# Autodesk Inventor assembly: ppe assembly
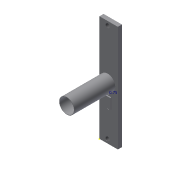
[picture p0: Inventor's stored thumbnail of the model, 180x180]
Saved by Autodesk Inventor 2019 (Build 230136000, 136)
## iProperties
Created: 2019-10-17
Part Number: ppe assembly
Document SubType Name: Assembly
Designer: Admin
Author: Admin
## Documents named in this file (5)
- C:\Users\Admin\Documents\ppe assembly.iam
- C:\Users\Admin\Documents\stand for pipe.ipt
- C:\Users\Admin\Documents\pipe.ipt
- C:\Users\Admin\Documents\SERVO MOTOR.ipt
- C:\Users\Admin\Documents\FLAPPER.ipt
## Components (4 placed, 4 different names)
1. stand for pipe:1 — Mate:1, Mate:2, Mate:3, Mate:4, Mate:5, Mate:6
2. pipe:1 — Mate:1, Mate:2, Mate:3
3. SERVO MOTOR:1 — Mate:4, Mate:5, Mate:6, Mate:7
4. FLAPPER:1 — Mate:7
## Relationships (7: Mate 7)
- Mate:1: stand for pipe:1 ↔ pipe:1
- Mate:2: stand for pipe:1 ↔ pipe:1
- Mate:3: stand for pipe:1 ↔ pipe:1
- Mate:4: stand for pipe:1 ↔ SERVO MOTOR:1
- Mate:5: stand for pipe:1 ↔ SERVO MOTOR:1
- Mate:6: stand for pipe:1 ↔ SERVO MOTOR:1
- Mate:7: SERVO MOTOR:1 ↔ FLAPPER:1
